# Autodesk Inventor assembly: Assembly1
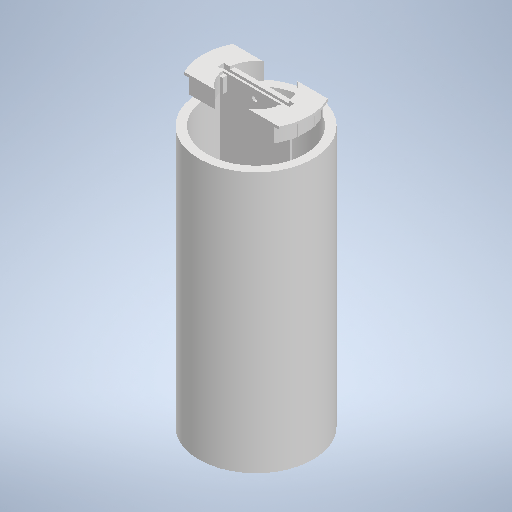
[picture p0: Inventor's stored thumbnail of the model, 512x512]
Saved by Autodesk Inventor 2025 (Build 290162010, 162A)
## iProperties
Created: 2024-06-20
Part Number: Assembly1
Document SubType Name: Assembly
Designer: vncnt
Author: vncnt
## Documents named in this file (4)
- C:\Users\vncnt\City Tech Dropbox\Vincent Ching\Community Sensor Lab Program\CAD\Air Quality Board Mount\Model 3\Assembly1.iam
- C:\Users\vncnt\City Tech Dropbox\Vincent Ching\Community Sensor Lab Program\CAD\Air Quality Board Mount\Model 2\Board.ipt
- C:\Users\vncnt\City Tech Dropbox\Vincent Ching\Community Sensor Lab Program\CAD\Air Quality Board Mount\pvc 3 in tube.ipt
- C:\Users\vncnt\City Tech Dropbox\Vincent Ching\Community Sensor Lab Program\CAD\Air Quality Board Mount\Model 3\Part2.ipt
## Components (3 placed, 3 different names)
1. pvc 3 in tube:1 — Insert:1
2. Part2:1 — Insert:1, Mate:1
3. Board:2 — Mate:1
## Relationships (2: Insert 1, Mate 1)
- Insert:1 (25.4 mm): pvc 3 in tube:1 ↔ Part2:1
- Mate:1: Part2:1 ↔ Board:2
